# Autodesk Inventor assembly: MGN block
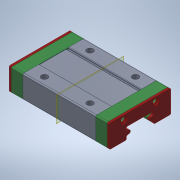
[picture p0: Inventor's stored thumbnail of the model, 180x180]
Saved by Autodesk Inventor 2020 (Build 240168000, 168)
## iProperties
Created: 2018-10-03
Part Number: MGN block
Document SubType Name: Assembly
Designer: LillaHunden
Mass: 8.35525 g
Surface Area: 68.7236 cm^2
Volume: 8.35525 cm^3
Density: 1 g/cm^3
Author: LillaHunden
## Documents named in this file (4)
- C:\Users\LillaHunden\Documents\Inventor\3dprinter\3dPrinter\Linear Rials import\MGN block.iam
- C:\Users\LillaHunden\Documents\Inventor\3dprinter\3dPrinter\Linear Rials import\Green End Cap.ipt
- C:\Users\LillaHunden\Documents\Inventor\3dprinter\3dPrinter\Linear Rials import\Main Block.ipt
- C:\Users\LillaHunden\Documents\Inventor\3dprinter\3dPrinter\Linear Rials import\Red End Cap.ipt
## Components (5 placed, 3 different names)
1. Green End Cap:1 — Mate:1, Flush:1, Flush:2, Mate:2, Flush:3, Flush:4
2. Main Block:1 — Mate:1, Flush:1, Flush:2, Mate:4, Flush:7, Flush:8
3. Red End Cap:1 — Mate:2, Flush:3, Flush:4, Symmetry:1
4. Green End Cap:2 — Mate:4, Flush:7, Flush:8
5. Red End Cap:2 — Symmetry:1
## Relationships (13: Flush 8, Mate 4, Symmetry 1)
- Mate:1: Green End Cap:1 ↔ Main Block:1
- Flush:1: Green End Cap:1 ↔ Main Block:1
- Flush:2: Green End Cap:1 ↔ Main Block:1
- Mate:2: Green End Cap:1 ↔ Red End Cap:1
- Flush:3: Green End Cap:1 ↔ Red End Cap:1
- Flush:4: Green End Cap:1 ↔ Red End Cap:1
- [Mate]: Green End Cap:2 ↔ Red End Cap:2
- [Flush]: Green End Cap:2 ↔ Red End Cap:2
- [Flush]: Green End Cap:2 ↔ Red End Cap:2
- Mate:4: Main Block:1 ↔ Green End Cap:2
- Flush:7: Main Block:1 ↔ Green End Cap:2
- Flush:8: Main Block:1 ↔ Green End Cap:2
- Symmetry:1: Red End Cap:1 ↔ Red End Cap:2
## Named parameters: d10_d7 = 0 mm, d11_d8 = 0 mm, d12_d9 = 0 mm
